# Autodesk Inventor assembly: StirnradUNDServo_MIR_MIR
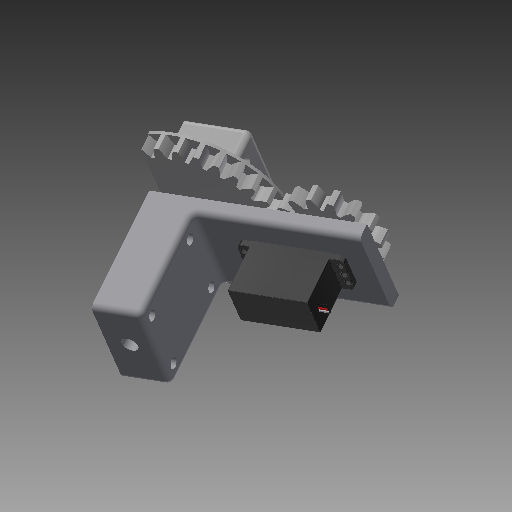
[picture p0: Inventor's stored thumbnail of the model, 512x512]
Saved by Autodesk Inventor 2018 (Build 220112000, 112)
## iProperties
Created: 2018-01-26
Part Number: StirnradUNDServo_MIR_MIR
Material: Generisch
Document SubType Name: Assembly
Designer: gchri
Mass: 191.612 g
Surface Area: 210.73 cm^2
Volume: 54.9428 cm^3
Density: 3.48748 g/cm^3
Author: gchri
## Documents named in this file (4)
- C:\Users\Chris\OneDrive\Development\Mohne\03_Konstruktion\StirnradUNDServo_MIR_MIR.iam
- C:\Users\Chris\OneDrive\Development\Mohne\03_Konstruktion\StirnradUNDServo\Konstruktions-Assistent\Stirnräder1_MIR_MIR.iam
- C:\Users\Chris\OneDrive\Development\Mohne\03_Konstruktion\servo_SM-S2309S_MIR_MIR.ipt
- C:\Users\Chris\OneDrive\Development\Mohne\03_Konstruktion\L-Halterung Servo_MIR1_MIR.ipt
## Components (3 placed, 3 different names)
1. Stirnräder1_MIR_MIR:1 [sub-assembly] — Passend:4, Passend:5
2. servo_SM-S2309S_MIR_MIR:1 — Passend:4, Passend:5, Passend:1, Passend:2, Passend:3
3. L-Halterung Servo_MIR1_MIR:1 — Passend:1, Passend:2, Passend:3
## Relationships (5: Mate 5)
- Passend:4 [Mate]: Stirnräder1_MIR_MIR:1 ↔ servo_SM-S2309S_MIR_MIR:1
- Passend:5 [Mate]: Stirnräder1_MIR_MIR:1 ↔ servo_SM-S2309S_MIR_MIR:1
- Passend:1 [Mate]: servo_SM-S2309S_MIR_MIR:1 ↔ L-Halterung Servo_MIR1_MIR:1
- Passend:2 [Mate]: servo_SM-S2309S_MIR_MIR:1 ↔ L-Halterung Servo_MIR1_MIR:1
- Passend:3 [Mate]: servo_SM-S2309S_MIR_MIR:1 ↔ L-Halterung Servo_MIR1_MIR:1
